# Autodesk Inventor assembly: DarkPoolFacility
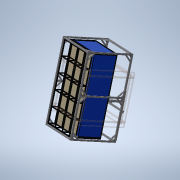
[picture p0: Inventor's stored thumbnail of the model, 180x180]
Saved by Autodesk Inventor 2022 (Build 260153000, 153)
## iProperties
Created: 2021-05-11
Part Number: DarkPoolFacility
Document SubType Name: Assembly
Designer: jamieson-bl
Author: jamieson-bl
## Documents named in this file (13)
- \\Mac\Home\Downloads\DarkPoolFacility.iam
- \\Mac\Home\Downloads\WinnipegPMTTestFacility-main\Room3L10.ipt
- \\Mac\Home\Downloads\WinnipegPMTTestFacility-main\iManikins\iMan\iMan.iam
- \\Mac\Home\Downloads\WinnipegPMTTestFacility-main\iManikins\iMandy\iMandy.iam
- \\Mac\Home\Downloads\WinnipegPMTTestFacility-main\Field Compensation Coils.iam
- \\Mac\Home\Downloads\WinnipegPMTTestFacility-main\ElectronicsRack.ipt
- \\Mac\Home\Downloads\WinnipegPMTTestFacility-main\CustomAquariumsStand.ipt
- \\Mac\Home\Downloads\WinnipegPMTTestFacility-main\CustomAquariumsTank.ipt
- \\Mac\Home\Downloads\WinnipegPMTTestFacility-main\gantry design\6060gantry.iam
- \\Mac\Home\Desktop\gantry design\standardbrackets\AIS2020\NBLUW8-60.iam
- \\Mac\Home\Desktop\gantry design\reinbracket\AIS2021\GFBL85050-250-SET.iam
- \\Mac\Home\Desktop\gantry design\rotary.ipt
- \\Mac\Home\Desktop\gantry design\steel-l-bracket-for-nema-23-stepper-motors.ipt
## Components (68 placed, 12 different names)
1. Room3L10:1 — Mate:2, Mate:3
2. iMan:1 [sub-assembly] — Mate:3
3. iMandy:1 [sub-assembly] — Mate:2
4. Field Compensation Coils:1 [sub-assembly] — Mate:5, Mate:6, Mate:7
5. ElectronicsRack:1
6. CustomAquariumsStand:1 — Mate:4, Flush:1, Flush:2, Mate:5, Mate:6, Flush:3, Mate:9
7. CustomAquariumsTank:1 — Mate:4, Flush:1, Flush:2, Mate:7, Mate:8
8. 6060gantry:1 [sub-assembly] — Flush:3, Mate:8, Mate:9, Mate:10, Flush:4, Mate:11, Mate:12, Mate:13, Flush:5, Mate:14, Mate:15, Flush:6, Mate:16, Mate:17, Flush:7, Mate:18, Mate:19, Flush:8, Mate:20, Mate:21, Flush:9, Mate:22, Mate:23, Flush:10, Mate:26, Mate:27, Flush:12, Mate:28, Flush:13, Flush:14, Mate:30, Mate:31, Flush:15, Mate:32, Mate:33, Flush:16, Mate:34, Mate:35, Flush:17, Mate:36, Mate:37, Flush:18, Mate:38, Mate:39, Flush:19, Mate:40, Mate:41, Flush:20, Mate:42, Mate:43, Flush:21, Mate:44, Mate:45, Flush:22, Mate:46, Mate:47, Flush:23, Mate:48, Mate:49, Flush:24, Mate:50, Mate:51, Flush:25, Mate:52, Mate:53, Flush:26, Mate:54, Mate:55, Flush:27, Mate:56, Mate:57, Flush:28, Mate:58, Mate:59, Flush:29, Mate:60, Mate:61, Flush:30, Mate:62, Mate:63, Flush:31, Mate:64, Mate:65, Flush:32, Mate:66, Mate:67, Flush:33, Mate:68, Mate:69, Flush:34, Mate:70, Mate:71, Flush:35, Mate:72, Mate:73, Flush:36, Mate:74, Mate:75, Flush:37, Mate:76, Mate:77, Flush:38, Mate:78, Mate:79, Flush:39, Mate:80, Mate:81, Flush:40, Mate:82, Mate:83, Flush:41, Mate:84, Mate:85, Flush:42, Mate:86, Mate:87, Flush:43, Mate:88, Mate:89, Flush:44, Mate:90, Mate:91, Flush:45, Mate:92, Mate:93, Flush:46, Mate:94, Mate:95, Flush:47, Mate:96, Mate:97, Flush:48, Mate:98, Mate:99, Flush:49, Mate:100, Mate:101, Flush:50, Mate:102, Mate:103, Flush:51, Mate:104, Mate:105, Flush:52, Mate:106, Mate:107, Flush:53, Mate:108, Mate:109, Flush:54, Mate:110, Mate:111, Flush:55, Mate:112, Mate:113, Flush:56, Mate:114, Mate:115, Flush:57, Mate:116, Mate:117, Flush:58, Mate:118, Mate:119, Flush:59, Mate:120, Mate:121, Flush:60, Mate:122, Mate:123, Flush:61, Mate:124, Mate:125, Flush:62, Mate:128, Flush:64, Flush:65, Mate:129, Flush:66, Mate:130, Mate:131, Flush:67, Flush:68
9. rotary:1 — Mate:28, Flush:13, Flush:14
10. steel-l-bracket-for-nema-23-stepper-motors:2 — Mate:131, Flush:67, Flush:68
11. steel-l-bracket-for-nema-23-stepper-motors:3 — Mate:128, Flush:64, Flush:65
12. steel-l-bracket-for-nema-23-stepper-motors:4 — Mate:129, Flush:66, Mate:130
13. NBLUW8-60:1 [sub-assembly] — Mate:10, Flush:4, Mate:11
14. NBLUW8-60:2 [sub-assembly] — Mate:14, Mate:15, Flush:6
15. NBLUW8-60:3 [sub-assembly] — Mate:12, Mate:13, Flush:5
16. NBLUW8-60:4 [sub-assembly] — Mate:16, Mate:17, Flush:7
17. NBLUW8-60:5 [sub-assembly] — Mate:20, Mate:21, Flush:9
18. NBLUW8-60:6 [sub-assembly] — Mate:18, Mate:19, Flush:8
19. NBLUW8-60:7 [sub-assembly] — Mate:76, Mate:77, Flush:38
20. NBLUW8-60:8 [sub-assembly] — Mate:74, Mate:75, Flush:37
21. NBLUW8-60:9 [sub-assembly] — Mate:78, Mate:79, Flush:39
22. NBLUW8-60:10 [sub-assembly] — Mate:82, Mate:83, Flush:41
23. NBLUW8-60:11 [sub-assembly] — Mate:80, Mate:81, Flush:40
24. NBLUW8-60:12 [sub-assembly] — Mate:84, Mate:85, Flush:42
25. NBLUW8-60:13 [sub-assembly] — Mate:86, Mate:87, Flush:43
26. NBLUW8-60:14 [sub-assembly] — Mate:88, Mate:89, Flush:44
27. NBLUW8-60:15 [sub-assembly] — Mate:90, Mate:91, Flush:45
28. NBLUW8-60:16 [sub-assembly] — Mate:92, Mate:93, Flush:46
29. NBLUW8-60:17 [sub-assembly] — Mate:100, Mate:101, Flush:50
30. NBLUW8-60:18 [sub-assembly] — Mate:104, Mate:105, Flush:52
31. NBLUW8-60:19 [sub-assembly] — Mate:102, Mate:103, Flush:51
32. NBLUW8-60:20 [sub-assembly] — Mate:94, Mate:95, Flush:47
33. NBLUW8-60:21 [sub-assembly] — Mate:96, Mate:97, Flush:48
34. NBLUW8-60:22 [sub-assembly] — Mate:98, Mate:99, Flush:49
35. NBLUW8-60:23 [sub-assembly] — Mate:116, Mate:117, Flush:58
36. NBLUW8-60:24 [sub-assembly] — Mate:114, Mate:115, Flush:57
37. NBLUW8-60:25 [sub-assembly] — Mate:112, Mate:113, Flush:56
38. NBLUW8-60:26 [sub-assembly] — Mate:106, Mate:107, Flush:53
39. NBLUW8-60:27 [sub-assembly] — Mate:108, Mate:109, Flush:54
40. NBLUW8-60:28 [sub-assembly] — Mate:110, Mate:111, Flush:55
41. NBLUW8-60:29 [sub-assembly] — Mate:118, Mate:119, Flush:59
42. NBLUW8-60:30 [sub-assembly] — Mate:120, Mate:121, Flush:60
43. NBLUW8-60:31 [sub-assembly] — Mate:124, Mate:125, Flush:62
44. NBLUW8-60:32 [sub-assembly] — Mate:122, Mate:123, Flush:61
45. GFBL85050-250-SET:1 [sub-assembly] — Mate:22, Mate:23, Flush:10
46. GFBL85050-250-SET:3 [sub-assembly] — Mate:26, Mate:27, Flush:12
47. GFBL85050-250-SET:4 [sub-assembly] — Mate:30, Mate:31, Flush:15
48. GFBL85050-250-SET:5 [sub-assembly] — Mate:36, Mate:37
49. GFBL85050-250-SET:6 [sub-assembly] — Mate:40, Mate:41, Flush:20
50. GFBL85050-250-SET:7 [sub-assembly] — Mate:38, Mate:39, Flush:19
51. GFBL85050-250-SET:8 [sub-assembly] — Mate:32, Mate:33, Flush:16
52. GFBL85050-250-SET:9 [sub-assembly] — Mate:34, Mate:35, Flush:17, Flush:18
53. GFBL85050-250-SET:10 [sub-assembly] — Mate:44, Mate:45, Flush:22
54. GFBL85050-250-SET:11 [sub-assembly] — Mate:42, Mate:43, Flush:21
55. GFBL85050-250-SET:12 [sub-assembly] — Mate:48, Mate:49, Flush:24
56. GFBL85050-250-SET:13 [sub-assembly] — Mate:46, Mate:47, Flush:23
57. GFBL85050-250-SET:14 [sub-assembly] — Mate:50, Mate:51, Flush:25
58. GFBL85050-250-SET:15 [sub-assembly] — Mate:52, Mate:53, Flush:26
59. GFBL85050-250-SET:16 [sub-assembly] — Mate:56, Mate:57, Flush:28
60. GFBL85050-250-SET:17 [sub-assembly] — Mate:54, Mate:55, Flush:27
61. GFBL85050-250-SET:18 [sub-assembly] — Mate:58, Mate:59, Flush:29
62. GFBL85050-250-SET:19 [sub-assembly] — Mate:62, Mate:63, Flush:31
63. GFBL85050-250-SET:20 [sub-assembly] — Mate:70, Mate:71, Flush:35
64. GFBL85050-250-SET:21 [sub-assembly] — Mate:68, Mate:69, Flush:34
65. GFBL85050-250-SET:22 [sub-assembly] — Mate:72, Mate:73, Flush:36
66. GFBL85050-250-SET:23 [sub-assembly] — Mate:60, Mate:61, Flush:30
67. GFBL85050-250-SET:24 [sub-assembly] — Mate:66, Mate:67, Flush:33
68. GFBL85050-250-SET:25 [sub-assembly] — Mate:64, Mate:65, Flush:32
## Relationships (191: Mate 125, Flush 66)
- Mate:2: Room3L10:1 ↔ iMandy:1
- Mate:3: Room3L10:1 ↔ iMan:1
- Mate:4: CustomAquariumsStand:1 ↔ CustomAquariumsTank:1
- Flush:1 (5.08 mm): CustomAquariumsStand:1 ↔ CustomAquariumsTank:1
- Flush:2: CustomAquariumsStand:1 ↔ CustomAquariumsTank:1
- Mate:5: Field Compensation Coils:1 ↔ CustomAquariumsStand:1
- Mate:6: Field Compensation Coils:1 ↔ CustomAquariumsStand:1
- Mate:7: Field Compensation Coils:1 ↔ CustomAquariumsTank:1
- Flush:3: CustomAquariumsStand:1 ↔ 6060gantry:1
- Mate:8 (50.8 mm): CustomAquariumsTank:1 ↔ 6060gantry:1
- Mate:9: CustomAquariumsStand:1 ↔ 6060gantry:1
- Mate:10: 6060gantry:1 ↔ NBLUW8-60:1
- Flush:4: 6060gantry:1 ↔ NBLUW8-60:1
- Mate:11: 6060gantry:1 ↔ NBLUW8-60:1
- Mate:12: 6060gantry:1 ↔ NBLUW8-60:3
- Mate:13: 6060gantry:1 ↔ NBLUW8-60:3
- Flush:5: 6060gantry:1 ↔ NBLUW8-60:3
- Mate:14: 6060gantry:1 ↔ NBLUW8-60:2
- Mate:15: 6060gantry:1 ↔ NBLUW8-60:2
- Flush:6: 6060gantry:1 ↔ NBLUW8-60:2
- Mate:16: 6060gantry:1 ↔ NBLUW8-60:4
- Mate:17: 6060gantry:1 ↔ NBLUW8-60:4
- Flush:7: 6060gantry:1 ↔ NBLUW8-60:4
- Mate:18: 6060gantry:1 ↔ NBLUW8-60:6
- Mate:19: 6060gantry:1 ↔ NBLUW8-60:6
- Flush:8: 6060gantry:1 ↔ NBLUW8-60:6
- Mate:20: 6060gantry:1 ↔ NBLUW8-60:5
- Mate:21: 6060gantry:1 ↔ NBLUW8-60:5
- Flush:9: 6060gantry:1 ↔ NBLUW8-60:5
- Mate:22: 6060gantry:1 ↔ GFBL85050-250-SET:1
- Mate:23: 6060gantry:1 ↔ GFBL85050-250-SET:1
- Flush:10: 6060gantry:1 ↔ GFBL85050-250-SET:1
- Mate:26: 6060gantry:1 ↔ GFBL85050-250-SET:3
- Mate:27: 6060gantry:1 ↔ GFBL85050-250-SET:3
- Flush:12: 6060gantry:1 ↔ GFBL85050-250-SET:3
- Mate:28: 6060gantry:1 ↔ rotary:1
- Flush:13: 6060gantry:1 ↔ rotary:1
- Flush:14: 6060gantry:1 ↔ rotary:1
- Mate:30: 6060gantry:1 ↔ GFBL85050-250-SET:4
- Mate:31: 6060gantry:1 ↔ GFBL85050-250-SET:4
- Flush:15: 6060gantry:1 ↔ GFBL85050-250-SET:4
- Mate:32: 6060gantry:1 ↔ GFBL85050-250-SET:8
- Mate:33: 6060gantry:1 ↔ GFBL85050-250-SET:8
- Flush:16: 6060gantry:1 ↔ GFBL85050-250-SET:8
- Mate:34: 6060gantry:1 ↔ GFBL85050-250-SET:9
- Mate:35: 6060gantry:1 ↔ GFBL85050-250-SET:9
- Flush:17: 6060gantry:1 ↔ GFBL85050-250-SET:9
- Mate:36: 6060gantry:1 ↔ GFBL85050-250-SET:5
- Mate:37: 6060gantry:1 ↔ GFBL85050-250-SET:5
- Flush:18: 6060gantry:1 ↔ GFBL85050-250-SET:9
- Mate:38: 6060gantry:1 ↔ GFBL85050-250-SET:7
- Mate:39: 6060gantry:1 ↔ GFBL85050-250-SET:7
- Flush:19: 6060gantry:1 ↔ GFBL85050-250-SET:7
- Mate:40: 6060gantry:1 ↔ GFBL85050-250-SET:6
- Mate:41: 6060gantry:1 ↔ GFBL85050-250-SET:6
- Flush:20: 6060gantry:1 ↔ GFBL85050-250-SET:6
- Mate:42: 6060gantry:1 ↔ GFBL85050-250-SET:11
- Mate:43: 6060gantry:1 ↔ GFBL85050-250-SET:11
- Flush:21: 6060gantry:1 ↔ GFBL85050-250-SET:11
- Mate:44: 6060gantry:1 ↔ GFBL85050-250-SET:10
- Mate:45: 6060gantry:1 ↔ GFBL85050-250-SET:10
- Flush:22: 6060gantry:1 ↔ GFBL85050-250-SET:10
- Mate:46: 6060gantry:1 ↔ GFBL85050-250-SET:13
- Mate:47: 6060gantry:1 ↔ GFBL85050-250-SET:13
- Flush:23: 6060gantry:1 ↔ GFBL85050-250-SET:13
- Mate:48: 6060gantry:1 ↔ GFBL85050-250-SET:12
- Mate:49: 6060gantry:1 ↔ GFBL85050-250-SET:12
- Flush:24: 6060gantry:1 ↔ GFBL85050-250-SET:12
- Mate:50: 6060gantry:1 ↔ GFBL85050-250-SET:14
- Mate:51: 6060gantry:1 ↔ GFBL85050-250-SET:14
- Flush:25: 6060gantry:1 ↔ GFBL85050-250-SET:14
- Mate:52: 6060gantry:1 ↔ GFBL85050-250-SET:15
- Mate:53: 6060gantry:1 ↔ GFBL85050-250-SET:15
- Flush:26: 6060gantry:1 ↔ GFBL85050-250-SET:15
- Mate:54: 6060gantry:1 ↔ GFBL85050-250-SET:17
- Mate:55: 6060gantry:1 ↔ GFBL85050-250-SET:17
- Flush:27: 6060gantry:1 ↔ GFBL85050-250-SET:17
- Mate:56: 6060gantry:1 ↔ GFBL85050-250-SET:16
- Mate:57: 6060gantry:1 ↔ GFBL85050-250-SET:16
- Flush:28: 6060gantry:1 ↔ GFBL85050-250-SET:16
- Mate:58: 6060gantry:1 ↔ GFBL85050-250-SET:18
- Mate:59: 6060gantry:1 ↔ GFBL85050-250-SET:18
- Flush:29: 6060gantry:1 ↔ GFBL85050-250-SET:18
- Mate:60: 6060gantry:1 ↔ GFBL85050-250-SET:23
- Mate:61: 6060gantry:1 ↔ GFBL85050-250-SET:23
- Flush:30: 6060gantry:1 ↔ GFBL85050-250-SET:23
- Mate:62: 6060gantry:1 ↔ GFBL85050-250-SET:19
- Mate:63: 6060gantry:1 ↔ GFBL85050-250-SET:19
- Flush:31: 6060gantry:1 ↔ GFBL85050-250-SET:19
- Mate:64: 6060gantry:1 ↔ GFBL85050-250-SET:25
- Mate:65: 6060gantry:1 ↔ GFBL85050-250-SET:25
- Flush:32: 6060gantry:1 ↔ GFBL85050-250-SET:25
- Mate:66: 6060gantry:1 ↔ GFBL85050-250-SET:24
- Mate:67: 6060gantry:1 ↔ GFBL85050-250-SET:24
- Flush:33: 6060gantry:1 ↔ GFBL85050-250-SET:24
- Mate:68: 6060gantry:1 ↔ GFBL85050-250-SET:21
- Mate:69: 6060gantry:1 ↔ GFBL85050-250-SET:21
- Flush:34: 6060gantry:1 ↔ GFBL85050-250-SET:21
- Mate:70: 6060gantry:1 ↔ GFBL85050-250-SET:20
- Mate:71: 6060gantry:1 ↔ GFBL85050-250-SET:20
- Flush:35: 6060gantry:1 ↔ GFBL85050-250-SET:20
- Mate:72: 6060gantry:1 ↔ GFBL85050-250-SET:22
- Mate:73: 6060gantry:1 ↔ GFBL85050-250-SET:22
- Flush:36: 6060gantry:1 ↔ GFBL85050-250-SET:22
- Mate:74: 6060gantry:1 ↔ NBLUW8-60:8
- Mate:75: 6060gantry:1 ↔ NBLUW8-60:8
- Flush:37: 6060gantry:1 ↔ NBLUW8-60:8
- Mate:76: 6060gantry:1 ↔ NBLUW8-60:7
- Mate:77: 6060gantry:1 ↔ NBLUW8-60:7
- Flush:38: 6060gantry:1 ↔ NBLUW8-60:7
- Mate:78: 6060gantry:1 ↔ NBLUW8-60:9
- Mate:79: 6060gantry:1 ↔ NBLUW8-60:9
- Flush:39: 6060gantry:1 ↔ NBLUW8-60:9
- Mate:80: 6060gantry:1 ↔ NBLUW8-60:11
- Mate:81: 6060gantry:1 ↔ NBLUW8-60:11
- Flush:40: 6060gantry:1 ↔ NBLUW8-60:11
- Mate:82: 6060gantry:1 ↔ NBLUW8-60:10
- Mate:83: 6060gantry:1 ↔ NBLUW8-60:10
- Flush:41: 6060gantry:1 ↔ NBLUW8-60:10
- Mate:84: 6060gantry:1 ↔ NBLUW8-60:12
- Mate:85: 6060gantry:1 ↔ NBLUW8-60:12
- Flush:42: 6060gantry:1 ↔ NBLUW8-60:12
- Mate:86: 6060gantry:1 ↔ NBLUW8-60:13
- Mate:87: 6060gantry:1 ↔ NBLUW8-60:13
- Flush:43: 6060gantry:1 ↔ NBLUW8-60:13
- Mate:88: 6060gantry:1 ↔ NBLUW8-60:14
- Mate:89: 6060gantry:1 ↔ NBLUW8-60:14
- Flush:44: 6060gantry:1 ↔ NBLUW8-60:14
- Mate:90: 6060gantry:1 ↔ NBLUW8-60:15
- Mate:91: 6060gantry:1 ↔ NBLUW8-60:15
- Flush:45: 6060gantry:1 ↔ NBLUW8-60:15
- Mate:92: 6060gantry:1 ↔ NBLUW8-60:16
- Mate:93: 6060gantry:1 ↔ NBLUW8-60:16
- Flush:46: 6060gantry:1 ↔ NBLUW8-60:16
- Mate:94: 6060gantry:1 ↔ NBLUW8-60:20
- Mate:95: 6060gantry:1 ↔ NBLUW8-60:20
- Flush:47: 6060gantry:1 ↔ NBLUW8-60:20
- Mate:96: 6060gantry:1 ↔ NBLUW8-60:21
- Mate:97: 6060gantry:1 ↔ NBLUW8-60:21
- Flush:48: 6060gantry:1 ↔ NBLUW8-60:21
- Mate:98: 6060gantry:1 ↔ NBLUW8-60:22
- Mate:99: 6060gantry:1 ↔ NBLUW8-60:22
- Flush:49: 6060gantry:1 ↔ NBLUW8-60:22
- Mate:100: 6060gantry:1 ↔ NBLUW8-60:17
- Mate:101: 6060gantry:1 ↔ NBLUW8-60:17
- Flush:50: 6060gantry:1 ↔ NBLUW8-60:17
- Mate:102: 6060gantry:1 ↔ NBLUW8-60:19
- Mate:103: 6060gantry:1 ↔ NBLUW8-60:19
- Flush:51: 6060gantry:1 ↔ NBLUW8-60:19
- Mate:104: 6060gantry:1 ↔ NBLUW8-60:18
- Mate:105: 6060gantry:1 ↔ NBLUW8-60:18
- Flush:52: 6060gantry:1 ↔ NBLUW8-60:18
- Mate:106: 6060gantry:1 ↔ NBLUW8-60:26
- Mate:107: 6060gantry:1 ↔ NBLUW8-60:26
- Flush:53: 6060gantry:1 ↔ NBLUW8-60:26
- Mate:108: 6060gantry:1 ↔ NBLUW8-60:27
- Mate:109: 6060gantry:1 ↔ NBLUW8-60:27
- Flush:54: 6060gantry:1 ↔ NBLUW8-60:27
- Mate:110: 6060gantry:1 ↔ NBLUW8-60:28
- Mate:111: 6060gantry:1 ↔ NBLUW8-60:28
- Flush:55: 6060gantry:1 ↔ NBLUW8-60:28
- Mate:112: 6060gantry:1 ↔ NBLUW8-60:25
- Mate:113: 6060gantry:1 ↔ NBLUW8-60:25
- Flush:56: 6060gantry:1 ↔ NBLUW8-60:25
- Mate:114: 6060gantry:1 ↔ NBLUW8-60:24
- Mate:115: 6060gantry:1 ↔ NBLUW8-60:24
- Flush:57: 6060gantry:1 ↔ NBLUW8-60:24
- Mate:116: 6060gantry:1 ↔ NBLUW8-60:23
- Mate:117: 6060gantry:1 ↔ NBLUW8-60:23
- Flush:58: 6060gantry:1 ↔ NBLUW8-60:23
- Mate:118: 6060gantry:1 ↔ NBLUW8-60:29
- Mate:119: 6060gantry:1 ↔ NBLUW8-60:29
- Flush:59: 6060gantry:1 ↔ NBLUW8-60:29
- Mate:120: 6060gantry:1 ↔ NBLUW8-60:30
- Mate:121: 6060gantry:1 ↔ NBLUW8-60:30
- Flush:60: 6060gantry:1 ↔ NBLUW8-60:30
- Mate:122: 6060gantry:1 ↔ NBLUW8-60:32
- Mate:123: 6060gantry:1 ↔ NBLUW8-60:32
- Flush:61: 6060gantry:1 ↔ NBLUW8-60:32
- Mate:124: 6060gantry:1 ↔ NBLUW8-60:31
- Mate:125: 6060gantry:1 ↔ NBLUW8-60:31
- Flush:62: 6060gantry:1 ↔ NBLUW8-60:31
- Mate:128: 6060gantry:1 ↔ steel-l-bracket-for-nema-23-stepper-motors:3
- Flush:64: 6060gantry:1 ↔ steel-l-bracket-for-nema-23-stepper-motors:3
- Flush:65: 6060gantry:1 ↔ steel-l-bracket-for-nema-23-stepper-motors:3
- Mate:129: 6060gantry:1 ↔ steel-l-bracket-for-nema-23-stepper-motors:4
- Flush:66: 6060gantry:1 ↔ steel-l-bracket-for-nema-23-stepper-motors:4
- Mate:130: 6060gantry:1 ↔ steel-l-bracket-for-nema-23-stepper-motors:4
- Mate:131: 6060gantry:1 ↔ steel-l-bracket-for-nema-23-stepper-motors:2
- Flush:67: 6060gantry:1 ↔ steel-l-bracket-for-nema-23-stepper-motors:2
- Flush:68: 6060gantry:1 ↔ steel-l-bracket-for-nema-23-stepper-motors:2
